# Autodesk Inventor assembly: Assembly2
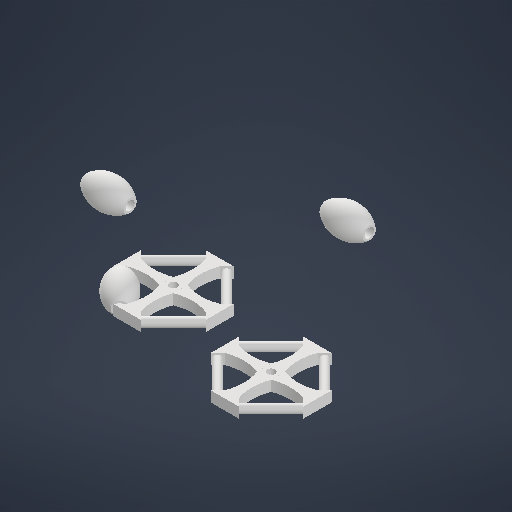
[picture p0: Inventor's stored thumbnail of the model, 512x512]
Saved by Autodesk Inventor 2026 (Build 300175000, 175)
## iProperties
Created: 2025-10-16
Part Number: Assembly2
Document SubType Name: Assembly
Designer: masak
Author: masak
## Documents named in this file (4)
- C:\Robohan\CAD\オムニ\Assembly2.iam
- C:\Robohan\CAD\オムニ\フレームD.ipt
- C:\Robohan\CAD\オムニ\フレームL.ipt
- C:\Robohan\CAD\オムニ\ホイール.ipt
## Components (7 placed, 3 different names)
1. フレームD:1 — 挿入:2, メイト:3
2. フレームL:1 — 挿入:1, 挿入:2, メイト:3
3. ホイール:1 — 挿入:1
4. ホイール:3
5. ホイール:4
6. フレームL:2 — メイト:2
7. フレームD:2 — メイト:2
## Relationships (4: Mate 2, Insert 2)
- メイト:2 [Mate]: フレームL:2 ↔ フレームD:2
- 挿入:1 [Insert] (0.5 mm): フレームL:1 ↔ ホイール:1
- 挿入:2 [Insert]: フレームD:1 ↔ フレームL:1
- メイト:3 [Mate]: フレームD:1 ↔ フレームL:1
